# Autodesk Inventor assembly: Multi-Cat
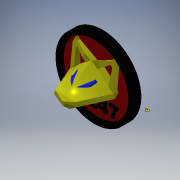
[picture p0: Inventor's stored thumbnail of the model, 180x180]
Saved by Autodesk Inventor 2016 (Build 200138000, 138)
## iProperties
Created: 2015-06-02
Part Number: Multi-Cat
Document SubType Name: Assembly
Designer: Spooner
Author: Spooner
## Documents named in this file (6)
- C:\Users\Spooner\Documents\Inventor\RoboCat Gen 2\Multi-Cat.iam
- C:\Users\Spooner\Documents\Inventor\RoboCat Gen 2\Background.ipt
- C:\Users\Spooner\Documents\Inventor\RoboCat Gen 2\Disk.ipt
- C:\Users\Spooner\Documents\Inventor\RoboCat Gen 2\Numbers.ipt
- C:\Users\Spooner\Documents\Inventor\RoboCat Gen 2\Cat.ipt
- C:\Users\Spooner\Documents\Inventor\RoboCat Gen 2\Eyes.ipt
## Components (5 placed, 5 different names)
1. Background:1 — Insert:1, Angle:2, Mate:3, Mate:4, Mate:5, Mate:6
2. Disk:1 — Mate:1, Mate:2, Insert:1, Angle:1, Angle:2, Tangent:1, Angle:3
3. Numbers:1 — Mate:3, Mate:4, Mate:5
4. Cat:1 — Mate:6, Tangent:1, Angle:3, Mate:7, Mate:8, Mate:9
5. Eyes:1 — Mate:7, Mate:8, Mate:9
## Relationships (14: Mate 9, Angle 3, Insert 1, Tangent 1)
- Mate:1: Disk:1
- Mate:2: Disk:1
- Insert:1: Background:1 ↔ Disk:1
- Angle:1 (0 deg): Disk:1
- Angle:2 (0 deg): Background:1 ↔ Disk:1
- Mate:3: Background:1 ↔ Numbers:1
- Mate:4: Background:1 ↔ Numbers:1
- Mate:5: Background:1 ↔ Numbers:1
- Mate:6: Background:1 ↔ Cat:1
- Tangent:1: Disk:1 ↔ Cat:1
- Angle:3 (0 deg): Disk:1 ↔ Cat:1
- Mate:7: Cat:1 ↔ Eyes:1
- Mate:8: Cat:1 ↔ Eyes:1
- Mate:9: Cat:1 ↔ Eyes:1
